# Autodesk Inventor assembly: AssemblyAll
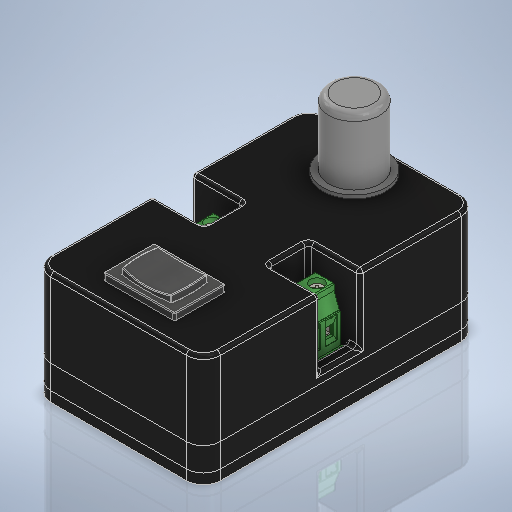
[picture p0: Inventor's stored thumbnail of the model, 512x512]
Saved by Autodesk Inventor 2025 (Build 290162010, 162A)
## iProperties
Created: 2025-11-03
Part Number: AssemblyAll
Document SubType Name: Assembly
Designer: João Vitor
Author: João Vitor
## Documents named in this file (8)
- C:\ProjectsOpenSource\SimpleAnalogDimmer\Inventor_Project\AssemblyAll.iam
- C:\ProjectsOpenSource\SimpleAnalogDimmer\Inventor_Project\LowerCase.ipt
- C:\ProjectsOpenSource\SimpleAnalogDimmer\Inventor_Project\PCB\DimmerCurso.iam
- C:\ProjectsOpenSource\SimpleAnalogDimmer\Inventor_Project\UpperCase.ipt
- C:\ProjectsOpenSource\SimpleAnalogDimmer\Inventor_Project\Knob.ipt
- C:\ProjectsOpenSource\SimpleAnalogDimmer\Inventor_Project\potansiyometre.ipt
- C:\ProjectsOpenSource\SimpleAnalogDimmer\Inventor_Project\Switch v1.ipt
- C:\ProjectsOpenSource\SimpleAnalogDimmer\Inventor_Project\SuportForWall.ipt
## Components (7 placed, 7 different names)
1. LowerCase:1 — Coincidente:1, Inserir:1, Coincidente:2, Coincidente:4, Coincidente:5, Coincidente:13, Coincidente:14, Coincidente:15
2. DimmerCurso:1 [sub-assembly] — Coincidente:1, Inserir:1, Coincidente:2
3. UpperCase:1 — Coincidente:4, Coincidente:5, Coincidente:7, Coincidente:8, Coincidente:10, Coincidente:11, Coincidente:12
4. Knob:1 — Coincidente:9, Inserir:2
5. potansiyometre:1 — Coincidente:7, Coincidente:8, Coincidente:9, Inserir:2
6. Switch v1:1 — Coincidente:10, Coincidente:11, Coincidente:12
7. SuportForWall:1 — Coincidente:13, Coincidente:14, Coincidente:15
## Relationships (15: Mate 13, Insert 2)
- Coincidente:1 [Mate]: LowerCase:1 ↔ DimmerCurso:1
- Inserir:1: LowerCase:1 ↔ DimmerCurso:1
- Coincidente:2 [Mate]: LowerCase:1 ↔ DimmerCurso:1
- Coincidente:4 [Mate]: LowerCase:1 ↔ UpperCase:1
- Coincidente:5 [Mate]: LowerCase:1 ↔ UpperCase:1
- Coincidente:7 [Mate] (0.5 mm): UpperCase:1 ↔ potansiyometre:1
- Coincidente:8 [Mate]: UpperCase:1 ↔ potansiyometre:1
- Coincidente:9 [Mate]: Knob:1 ↔ potansiyometre:1
- Inserir:2: Knob:1 ↔ potansiyometre:1
- Coincidente:10 [Mate]: UpperCase:1 ↔ Switch v1:1
- Coincidente:11 [Mate] (1.1 mm): UpperCase:1 ↔ Switch v1:1
- Coincidente:12 [Mate]: UpperCase:1 ↔ Switch v1:1
- Coincidente:13 [Mate]: LowerCase:1 ↔ SuportForWall:1
- Coincidente:14 [Mate]: LowerCase:1 ↔ SuportForWall:1
- Coincidente:15 [Mate]: LowerCase:1 ↔ SuportForWall:1
